# Autodesk Inventor assembly: RoboCats
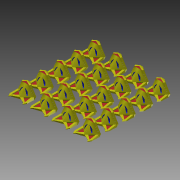
[picture p0: Inventor's stored thumbnail of the model, 180x180]
Saved by Autodesk Inventor 2014 (Build 180170000, 170)
## iProperties
Created: 2014-01-20
Part Number: RoboCats
Document SubType Name: Assembly
Designer: Spooner
Author: Spooner
## Documents named in this file (2)
- C:\Users\Spooner\Documents\Cubify\RoboCat\RoboCats.iam
- C:\Users\Spooner\Documents\Cubify\RoboCat\roboCat1.ipt
## Components (20 placed, 1 different names)
1. roboCat1:1
2. roboCat1:2 — Flush:1
3. roboCat1:3 — Flush:1, Flush:2
4. roboCat1:4 — Flush:2, Flush:3
5. roboCat1:5 — Flush:3
6. roboCat1:6
7. roboCat1:7
8. roboCat1:8
9. roboCat1:9
10. roboCat1:10
11. roboCat1:11
12. roboCat1:12
13. roboCat1:13
14. roboCat1:14
15. roboCat1:15
16. roboCat1:16
17. roboCat1:17
18. roboCat1:18
19. roboCat1:19
20. roboCat1:20
## Component patterns: (4 elements, first: roboCat1:1 + roboCat1:2 + roboCat1:3 + roboCat1:4 + roboCat1:5)
## Relationships (3: Flush 3)
- Flush:1: roboCat1:2 ↔ roboCat1:3
- Flush:2: roboCat1:3 ↔ roboCat1:4
- Flush:3: roboCat1:4 ↔ roboCat1:5
